# Autodesk Inventor assembly: A2_PongBoy
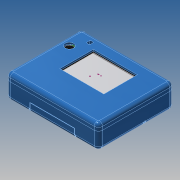
[picture p0: Inventor's stored thumbnail of the model, 180x180]
Saved by Autodesk Inventor 2020.2 (Build 242310000, 310)
## iProperties
Created: 2021-08-30
Part Number: A2_PongBoy
Document SubType Name: Assembly
Designer: Samy Francelet
Author: Samy Francelet
## Documents named in this file (6)
- D:\work\PongBoy\0400_Mechanical\A2_PongBoy.iam
- D:\work\PongBoy\0400_Mechanical\P1_BottomCase.ipt
- D:\work\PongBoy\0400_Mechanical\A1_PCB.iam
- D:\work\PongBoy\0400_Mechanical\P3_BatteriesTray.ipt
- D:\work\PongBoy\0400_Mechanical\P2_TopCase.ipt
- D:\work\PongBoy\0400_Mechanical\P4_Stylet.ipt
## Components (5 placed, 5 different names)
1. P1_BottomCase:1 — Placage:1, Placage:2, Placage:4, Placage:5, Affleurement:1, Placage:7, Affleurement:2, Affleurement:3, Placage:8, Cylindrique:1, Affleurement:4, Placage:9
2. A1_PCB:1 [sub-assembly] — Placage:1, Placage:2, Placage:7
3. P3_BatteriesTray:1 — Placage:4, Placage:5, Affleurement:1
4. P2_TopCase:1 — Affleurement:2, Affleurement:3, Placage:8
5. P4_Stylet:1 — Cylindrique:1, Affleurement:4, Placage:9
## Relationships (12: Mate 7, Flush 4, CylindricalJoint 1)
- Placage:1 [Mate]: P1_BottomCase:1 ↔ A1_PCB:1
- Placage:2 [Mate]: P1_BottomCase:1 ↔ A1_PCB:1
- Placage:4 [Mate]: P1_BottomCase:1 ↔ P3_BatteriesTray:1
- Placage:5 [Mate]: P1_BottomCase:1 ↔ P3_BatteriesTray:1
- Affleurement:1 [Flush]: P1_BottomCase:1 ↔ P3_BatteriesTray:1
- Placage:7 [Mate]: P1_BottomCase:1 ↔ A1_PCB:1
- Affleurement:2 [Flush]: P1_BottomCase:1 ↔ P2_TopCase:1
- Affleurement:3 [Flush]: P1_BottomCase:1 ↔ P2_TopCase:1
- Placage:8 [Mate]: P1_BottomCase:1 ↔ P2_TopCase:1
- Cylindrique:1: P1_BottomCase:1 ↔ P4_Stylet:1
- Affleurement:4 [Flush] (0.5 mm): P1_BottomCase:1 ↔ P4_Stylet:1
- Placage:9 [Mate]: P1_BottomCase:1 ↔ P4_Stylet:1
